# Autodesk Inventor assembly: Casioassembly2
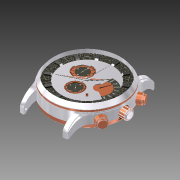
[picture p0: Inventor's stored thumbnail of the model, 180x180]
Saved by Autodesk Inventor 2012 (Build 160160000, 160)
## iProperties
Created: 2013-09-09
Part Number: Casioassembly2
Document SubType Name: Assembly
Designer: Satellite
Author: Satellite
## Documents named in this file (5)
- C:\Users\Satellite\Desktop\Casioassembly2.iam
- C:\Users\Satellite\Desktop\Casiobody.ipt
- C:\Users\Satellite\Desktop\Casioassembly1.iam
- C:\Users\Satellite\Desktop\Casiosidenob.ipt
- C:\Users\Satellite\Desktop\Casiomiddlenob.ipt
## Components (5 placed, 4 different names)
1. Casiobody:1 — Insert:1, Flush:1, Insert:2, Insert:3, Insert:4
2. Casioassembly1:1 [sub-assembly] — Insert:1, Flush:1
3. Casiosidenob:1 — Insert:3
4. Casiomiddlenob:1 — Insert:4
5. Casiosidenob:2 — Insert:2
## Relationships (5: Insert 4, Flush 1)
- Insert:1: Casiobody:1 ↔ Casioassembly1:1
- Flush:1: Casiobody:1 ↔ Casioassembly1:1
- Insert:2: Casiobody:1 ↔ Casiosidenob:2
- Insert:3: Casiobody:1 ↔ Casiosidenob:1
- Insert:4: Casiobody:1 ↔ Casiomiddlenob:1
